# Autodesk Inventor assembly: Falcon with Gearbox 2 stage_MIR_MIR
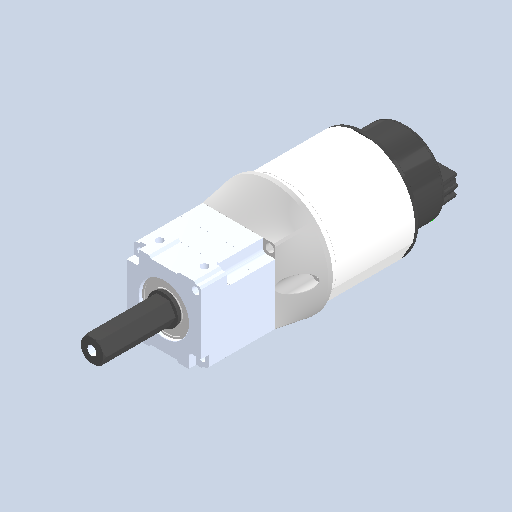
[picture p0: Inventor's stored thumbnail of the model, 512x512]
Saved by Autodesk Inventor 2023 (Build 270158000, 158)
## iProperties
Created: 2023-02-06
Part Number: Falcon with Gearbox 2 stage_MIR_MIR
Document SubType Name: Assembly
Designer: Gabriel - T3 CAD
Author: Gabriel - T3 CAD
## Documents named in this file (4)
- C:\Users\Gabriel - T3 CAD\Documents\GitHub\T3-CAD\Stock\Motors and Gearboxes\Falcon with Gearbox 2 stage_MIR_MIR.iam
- C:\Users\Gabriel - T3 CAD\Documents\GitHub\T3-CAD\Stock\Electronics\Falcon 500_MIR_MIR.ipt
- C:\Users\Gabriel - T3 CAD\Documents\GitHub\T3-CAD\Stock\Motors and Gearboxes\VersaPlanetary CIM Adapter (217-4018)_MIR_MIR.ipt
- C:\Users\Gabriel - T3 CAD\Documents\GitHub\T3-CAD\Stock\Versa System\VersaPlanetary\VersaPlanetary v2 Two Stage 100_1 with BAG _Simplify_1_MIR_MIR.ipt
## Components (3 placed, 3 different names)
1. Falcon 500_MIR_MIR:1 — Rotational:1, Rotational:2
2. VersaPlanetary CIM Adapter (217-4018)_MIR_MIR:1 — Rotational:1, Rotational:2, Rotational:3, Rotational:4
3. VersaPlanetary v2 Two Stage 100_1 with BAG _Simplify_1_MIR_MIR:1 — Rotational:3, Rotational:4
## Relationships (4: RevoluteJoint 4)
- Rotational:1 [RevoluteJoint]: Falcon 500_MIR_MIR:1 ↔ VersaPlanetary CIM Adapter (217-4018)_MIR_MIR:1
- Rotational:2 [RevoluteJoint]: Falcon 500_MIR_MIR:1 ↔ VersaPlanetary CIM Adapter (217-4018)_MIR_MIR:1
- Rotational:3 [RevoluteJoint]: VersaPlanetary CIM Adapter (217-4018)_MIR_MIR:1 ↔ VersaPlanetary v2 Two Stage 100_1 with BAG _Simplify_1_MIR_MIR:1
- Rotational:4 [RevoluteJoint]: VersaPlanetary CIM Adapter (217-4018)_MIR_MIR:1 ↔ VersaPlanetary v2 Two Stage 100_1 with BAG _Simplify_1_MIR_MIR:1
